# Autodesk Inventor assembly: roughDraft-12inchBase
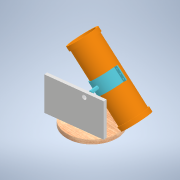
[picture p0: Inventor's stored thumbnail of the model, 180x180]
Saved by Autodesk Inventor 2021 (Build 250183000, 183)
## iProperties
Created: 2020-07-01
Part Number: roughDraft-12inchBase
Document SubType Name: Assembly
Designer: robst
Author: robst
## Documents named in this file (5)
- C:\git\CAD-Development\robSteele\ShapeWays\TelescopeProjects\TelescopeMount\roughDraft-12inchBase.iam
- C:\git\CAD-Development\robSteele\ShapeWays\TelescopeProjects\TelescopeMount\base-12-inch-diameter.ipt
- C:\git\CAD-Development\robSteele\ShapeWays\TelescopeProjects\TelescopeMount\sideSupportFor12inchBase.ipt
- C:\git\CAD-Development\robSteele\ShapeWays\TelescopeProjects\TelescopeMount\tubeBracketV02.ipt
- C:\git\CAD-Development\robSteele\ShapeWays\TelescopeProjects\TelescopeMount\telescopeTube.ipt
## Components (4 placed, 4 different names)
1. base-12-inch-diameter:1 — Flush:1, Flush:2
2. sideSupportFor12inchBase:1 — Flush:1, Flush:2, Insert:1
3. tubeBracketV02:1 — Insert:1, Flush:3, Flush:4, Mate:1
4. telescopeTube:1 — Flush:3, Flush:4, Mate:1
## Relationships (6: Flush 4, Insert 1, Mate 1)
- Flush:1: base-12-inch-diameter:1 ↔ sideSupportFor12inchBase:1
- Flush:2: base-12-inch-diameter:1 ↔ sideSupportFor12inchBase:1
- Insert:1 (25.4 mm): sideSupportFor12inchBase:1 ↔ tubeBracketV02:1
- Flush:3: tubeBracketV02:1 ↔ telescopeTube:1
- Flush:4: tubeBracketV02:1 ↔ telescopeTube:1
- Mate:1: tubeBracketV02:1 ↔ telescopeTube:1
